# Autodesk Inventor assembly: Frame
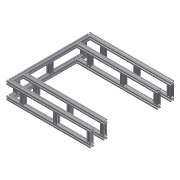
[picture p0: Inventor's stored thumbnail of the model, 180x180]
Saved by Autodesk Inventor 2011 (Build 150239000, 239)
## iProperties
Created: 2013-10-03
Part Number: Frame
Document SubType Name: Assembly
Designer: Family Room
Author: Family Room
## Documents named in this file (5)
- J:\FTC\Frame.iam
- J:\FTC\Back.ipt
- J:\FTC\Long side.ipt
- J:\FTC\vertical.ipt
- J:\FTC\short side.ipt
## Components (25 placed, 4 different names)
1. Back:1 — Mate:1, Flush:1, Flush:2, Mate:2, Flush:3, Flush:4, Mate:5, Flush:9, Mate:7, Flush:10, Flush:16, Mate:20, Flush:30, Mate:21, Flush:32, Mate:22, Flush:34, Flush:40, Flush:41, Flush:43
2. Back:2 — Flush:40, Mate:25, Flush:41
3. Long side:1 — Mate:1, Flush:1, Flush:2, Mate:3, Flush:5, Flush:6, Mate:6, Mate:11, Flush:15, Mate:15, Flush:23, Flush:31, Flush:33
4. Long side:2 — Mate:2, Flush:3, Flush:4, Mate:4, Flush:7, Flush:8, Mate:8, Mate:14, Flush:21, Mate:19, Flush:28, Flush:35, Flush:45
5. vertical:1 — Mate:3, Flush:5, Flush:6, Mate:16
6. vertical:2 — Mate:4, Flush:7, Flush:8, Mate:27, Flush:44
7. short side:1 — Mate:5, Flush:9, Mate:6, Mate:9, Flush:11, Flush:12, Mate:12, Flush:17, Mate:17, Flush:24, Flush:37
8. short side:2 — Mate:7, Flush:10, Mate:8, Mate:10, Flush:13, Flush:14, Mate:13, Flush:19, Mate:18, Flush:26, Flush:39
9. vertical:3 — Mate:9, Flush:11, Flush:12, Mate:23, Flush:36
10. vertical:4 — Mate:10, Flush:13, Flush:14, Mate:24, Flush:38
11. vertical:5 — Mate:11, Flush:15, Flush:16, Flush:18, Mate:26, Flush:42
12. vertical:6 — Mate:14, Flush:21, Flush:22
13. vertical:7 — Mate:12, Flush:17, Flush:18, Flush:20
14. vertical:8 — Mate:13, Flush:19, Flush:20, Flush:22
15. vertical:9 — Mate:15, Flush:23, Mate:16, Flush:25
16. vertical:10 — Mate:18, Flush:26, Flush:27, Flush:29
17. vertical:11 — Mate:17, Flush:24, Flush:25, Flush:27
18. vertical:12 — Mate:19, Flush:28, Flush:29
19. vertical:13 — Mate:21, Flush:32, Flush:33
20. vertical:14 — Mate:20, Flush:30, Flush:31
21. vertical:15 — Mate:22, Flush:34, Flush:35, Mate:25
22. short side:3 — Mate:23, Flush:36, Flush:37
23. short side:4 — Mate:24, Flush:38, Flush:39
24. Long side:3 — Mate:26, Flush:42, Flush:43
25. Long side:4 — Mate:27, Flush:44, Flush:45
## Relationships (72: Flush 45, Mate 27)
- Mate:1: Back:1 ↔ Long side:1
- Flush:1: Back:1 ↔ Long side:1
- Flush:2: Back:1 ↔ Long side:1
- Mate:2: Back:1 ↔ Long side:2
- Flush:3: Back:1 ↔ Long side:2
- Flush:4: Back:1 ↔ Long side:2
- Mate:3: Long side:1 ↔ vertical:1
- Flush:5: Long side:1 ↔ vertical:1
- Flush:6: Long side:1 ↔ vertical:1
- Mate:4: Long side:2 ↔ vertical:2
- Flush:7: Long side:2 ↔ vertical:2
- Flush:8: Long side:2 ↔ vertical:2
- Mate:5: Back:1 ↔ short side:1
- Flush:9: Back:1 ↔ short side:1
- Mate:6 (50.8 mm): Long side:1 ↔ short side:1
- Mate:7: Back:1 ↔ short side:2
- Flush:10: Back:1 ↔ short side:2
- Mate:8 (50.8 mm): Long side:2 ↔ short side:2
- Mate:9: short side:1 ↔ vertical:3
- Flush:11: short side:1 ↔ vertical:3
- Flush:12: short side:1 ↔ vertical:3
- Mate:10: short side:2 ↔ vertical:4
- Flush:13: short side:2 ↔ vertical:4
- Flush:14: short side:2 ↔ vertical:4
- Mate:11: Long side:1 ↔ vertical:5
- Flush:15: Long side:1 ↔ vertical:5
- Flush:16 (70.8 mm): Back:1 ↔ vertical:5
- Mate:12: short side:1 ↔ vertical:7
- Flush:17: short side:1 ↔ vertical:7
- Flush:18: vertical:5 ↔ vertical:7
- Mate:13: short side:2 ↔ vertical:8
- Flush:19: short side:2 ↔ vertical:8
- Flush:20: vertical:7 ↔ vertical:8
- Mate:14: Long side:2 ↔ vertical:6
- Flush:21: Long side:2 ↔ vertical:6
- Flush:22: vertical:6 ↔ vertical:8
- Mate:15: Long side:1 ↔ vertical:9
- Flush:23: Long side:1 ↔ vertical:9
- Mate:16 (156.8526 mm): vertical:1 ↔ vertical:9
- Mate:17: short side:1 ↔ vertical:11
- Flush:24: short side:1 ↔ vertical:11
- Flush:25: vertical:9 ↔ vertical:11
- Mate:18: short side:2 ↔ vertical:10
- Flush:26: short side:2 ↔ vertical:10
- Flush:27: vertical:10 ↔ vertical:11
- Mate:19: Long side:2 ↔ vertical:12
- Flush:28: Long side:2 ↔ vertical:12
- Flush:29: vertical:10 ↔ vertical:12
- Mate:20: Back:1 ↔ vertical:14
- Flush:30: Back:1 ↔ vertical:14
- Flush:31 (212.25 mm): Long side:1 ↔ vertical:14
- Mate:21: Back:1 ↔ vertical:13
- Flush:32: Back:1 ↔ vertical:13
- Flush:33 (35.4 mm): Long side:1 ↔ vertical:13
- Mate:22: Back:1 ↔ vertical:15
- Flush:34: Back:1 ↔ vertical:15
- Flush:35 (-35.4 mm): Long side:2 ↔ vertical:15
- Mate:23: vertical:3 ↔ short side:3
- Flush:36: vertical:3 ↔ short side:3
- Flush:37: short side:1 ↔ short side:3
- Mate:24: vertical:4 ↔ short side:4
- Flush:38: vertical:4 ↔ short side:4
- Flush:39: short side:2 ↔ short side:4
- Flush:40: Back:1 ↔ Back:2
- Mate:25: Back:2 ↔ vertical:15
- Flush:41: Back:1 ↔ Back:2
- Mate:26: vertical:5 ↔ Long side:3
- Flush:42: vertical:5 ↔ Long side:3
- Flush:43: Back:1 ↔ Long side:3
- Mate:27: vertical:2 ↔ Long side:4
- Flush:44: vertical:2 ↔ Long side:4
- Flush:45: Long side:2 ↔ Long side:4
